# Autodesk Inventor assembly: wheel_assembly
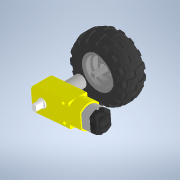
[picture p0: Inventor's stored thumbnail of the model, 180x180]
Saved by Autodesk Inventor 2020.3 (Build 243373000, 373)
## iProperties
Created: 2021-08-07
Part Number: wheel_assembly
Document SubType Name: Assembly
Designer: 0x6f736f646f
Author: 0x6f736f646f
## Documents named in this file (6)
- C:\Users\Public\D\Desktop\Trash\Design-of-an-Automatic-Nurse-Assitant\src\Design\wheel_assembly.iam
- C:\Users\Public\D\Desktop\Trash\Design-of-an-Automatic-Nurse-Assitant\src\Design\motor.ipt
- C:\Users\Public\D\Desktop\Trash\Design-of-an-Automatic-Nurse-Assitant\src\Design\wheel.ipt
- C:\Users\Public\D\Desktop\Trash\Design-of-an-Automatic-Nurse-Assitant\src\Design\wheel_bar.ipt
- C:\Users\Public\D\Desktop\Trash\Design-of-an-Automatic-Nurse-Assitant\src\Design\wheel_rim.ipt
- C:\Users\Public\D\Desktop\Trash\Design-of-an-Automatic-Nurse-Assitant\src\Design\wheel_tube.ipt
## Components (5 placed, 5 different names)
1. motor:1 — Mate:1, Mate:2
2. wheel:1 — Mate:3, Mate:4
3. wheel_bar:1 — Flush:1, Mate:5, Mate:6, Mate:7
4. wheel_rim:1 — Mate:3, Mate:4, Flush:1, Mate:5, Mate:6
5. wheel_tube:1 — Mate:1, Mate:2, Mate:7
## Relationships (8: Mate 7, Flush 1)
- Mate:1: motor:1 ↔ wheel_tube:1
- Mate:2: motor:1 ↔ wheel_tube:1
- Mate:3: wheel:1 ↔ wheel_rim:1
- Mate:4: wheel:1 ↔ wheel_rim:1
- Flush:1: wheel_bar:1 ↔ wheel_rim:1
- Mate:5: wheel_bar:1 ↔ wheel_rim:1
- Mate:6: wheel_bar:1 ↔ wheel_rim:1
- Mate:7: wheel_bar:1 ↔ wheel_tube:1
